# Autodesk Inventor assembly: Sheet_Assembly
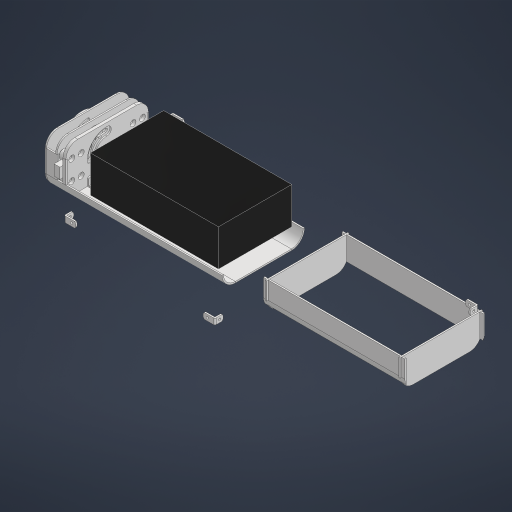
[picture p0: Inventor's stored thumbnail of the model, 512x512]
Saved by Autodesk Inventor 2024 (Build 280153000, 153)
## iProperties
Created: 2024-02-24
Part Number: Sheet_Assembly
Document SubType Name: Assembly
Designer: calvi
Author: calvi
## Documents named in this file (15)
- C:\Users\calvi\OneDrive\Robocup Rescue\Chassis\Battery Drawer\Sheet_Assembly.iam
- C:\Users\calvi\OneDrive\Robocup Rescue\Chassis\Battery Drawer\Sheet.ipt
- C:\Users\calvi\OneDrive\Robocup Rescue\Chassis\Battery Drawer\Plate_middle.ipt
- C:\Users\calvi\OneDrive\Robocup Rescue\Chassis\Battery Drawer\Plate_back.ipt
- C:\Users\calvi\OneDrive\Robocup Rescue\Chassis\Battery Drawer\Crank.ipt
- C:\Users\calvi\OneDrive\Robocup Rescue\Chassis\Battery Drawer\Peg.ipt
- C:\Users\calvi\OneDrive\Robocup Rescue\Chassis\Battery Drawer\Handle.ipt
- C:\Users\calvi\OneDrive\Robocup Rescue\Chassis\Battery Drawer\Slider1.ipt
- Slider1.ipt
- C:\Users\calvi\OneDrive\Robocup Rescue\Chassis\Battery Drawer\Slider2.ipt
- C:\Users\calvi\OneDrive\Robocup Rescue\Chassis\Battery Drawer\6389K345_Light Duty Dry-Running Nylon Sleeve Bearing\6389K345_Light Duty Dry-Running Nylon Sleeve Bearing.ipt
- C:\Users\calvi\OneDrive\Robocup Rescue\Chassis\Battery Drawer\Zinc-Plated Steel Corner Bracket3\Zinc-Plated Steel Corner Bracket3.ipt
- C:\Users\calvi\OneDrive\Robocup Rescue\Chassis\Electronics Box\EBox-Parts\MainBattery.ipt
- MainBattery-E.ipt
- C:\Users\calvi\OneDrive\Robocup Rescue\Chassis\Battery Drawer\BatteryHolder\Battery_Holder_Assembly.iam
## Components (27 placed, 12 different names)
1. Sheet:1 — Mate:1, Mate:2, Mate:3, Mate:4, Mate:5, Mate:10, Mate:12, Mate:13, Mate:15, Rotational:9, Mate:18, Mate:19, Mate:20, Mate:21, Mate:27, Mate:28
2. Plate_middle:1 — Mate:1, Mate:2, Mate:3, Rotational:1, Rotational:2, Rotational:3, Rotational:4, Rotational:5, Rotational:6, Rotational:7, Rotational:8, Mate:6, Flush:1, Mate:7, Flush:2, Mate:16, Mate:17
3. Plate_back:1 — Mate:4, Mate:5, Rigid:1, Mate:11, Mate:14
4. Crank:1 — Rigid:10, Rotational:9, Cylindrical:1, Cylindrical:2
5. Peg:1 — Slider:2, Cylindrical:1
6. Peg:2 — Slider:1, Cylindrical:2
7. Handle:1 — Rigid:10
8. Slider1:1 — Mate:6, Flush:1, Slider:2
9. Slider2:1 — Mate:7, Flush:2, Slider:1
10. MainBattery-E:2 — Mate:25
11. Battery_Holder_Assembly:1 [sub-assembly] — Mate:25, Mate:27, Mate:28, Mate:29, Mate:30
12. Zinc-Plated Steel Corner Bracket3:5
13. Zinc-Plated Steel Corner Bracket3:6
14. Zinc-Plated Steel Corner Bracket3:7
15. Zinc-Plated Steel Corner Bracket3:8 — Mate:29, Mate:30
16. 6389K345_Light Duty Dry-Running Nylon Sleeve Bearing:8 — Rotational:8
17. 6389K345_Light Duty Dry-Running Nylon Sleeve Bearing:7 — Rotational:7
18. 6389K345_Light Duty Dry-Running Nylon Sleeve Bearing:6 — Rotational:5
19. 6389K345_Light Duty Dry-Running Nylon Sleeve Bearing:5 — Rotational:6, Rigid:1
20. 6389K345_Light Duty Dry-Running Nylon Sleeve Bearing:4 — Rotational:4
21. 6389K345_Light Duty Dry-Running Nylon Sleeve Bearing:3 — Rotational:3
22. 6389K345_Light Duty Dry-Running Nylon Sleeve Bearing:2 — Rotational:2
23. 6389K345_Light Duty Dry-Running Nylon Sleeve Bearing:1 — Rotational:1
24. Zinc-Plated Steel Corner Bracket3:4 — Mate:17, Mate:18, Mate:21
25. Zinc-Plated Steel Corner Bracket3:3 — Mate:16, Mate:19, Mate:20
26. Zinc-Plated Steel Corner Bracket3:2 — Mate:13, Mate:14, Mate:15
27. Zinc-Plated Steel Corner Bracket3:1 — Mate:10, Mate:11, Mate:12
## Relationships (41: Mate 24, RevoluteJoint 9, Flush 2, WeldJoint 2, TranslationJoint 2, CylindricalJoint 2)
- Mate:1: Sheet:1 ↔ Plate_middle:1
- Mate:2: Sheet:1 ↔ Plate_middle:1
- Mate:3 (19.177 mm): Sheet:1 ↔ Plate_middle:1
- Mate:4: Sheet:1 ↔ Plate_back:1
- Mate:5: Sheet:1 ↔ Plate_back:1
- Rotational:1 [RevoluteJoint]: Plate_middle:1 ↔ 6389K345_Light Duty Dry-Running Nylon Sleeve Bearing:1
- Rotational:2 [RevoluteJoint]: Plate_middle:1 ↔ 6389K345_Light Duty Dry-Running Nylon Sleeve Bearing:2
- Rotational:3 [RevoluteJoint]: Plate_middle:1 ↔ 6389K345_Light Duty Dry-Running Nylon Sleeve Bearing:3
- Rotational:4 [RevoluteJoint]: Plate_middle:1 ↔ 6389K345_Light Duty Dry-Running Nylon Sleeve Bearing:4
- Rotational:5 [RevoluteJoint]: Plate_middle:1 ↔ 6389K345_Light Duty Dry-Running Nylon Sleeve Bearing:6
- Rotational:6 [RevoluteJoint]: Plate_middle:1 ↔ 6389K345_Light Duty Dry-Running Nylon Sleeve Bearing:5
- Rotational:7 [RevoluteJoint]: Plate_middle:1 ↔ 6389K345_Light Duty Dry-Running Nylon Sleeve Bearing:7
- Rotational:8 [RevoluteJoint]: Plate_middle:1 ↔ 6389K345_Light Duty Dry-Running Nylon Sleeve Bearing:8
- Mate:6: Plate_middle:1 ↔ Slider1:1
- Flush:1 (-11.43 mm): Plate_middle:1 ↔ Slider1:1
- Mate:7: Plate_middle:1 ↔ Slider2:1
- Flush:2 (-11.43 mm): Plate_middle:1 ↔ Slider2:1
- Rigid:1 [WeldJoint]: Plate_back:1 ↔ 6389K345_Light Duty Dry-Running Nylon Sleeve Bearing:5
- Mate:10: Sheet:1 ↔ Zinc-Plated Steel Corner Bracket3:1
- Mate:11: Plate_back:1 ↔ Zinc-Plated Steel Corner Bracket3:1
- Mate:12 (43.18 mm): Sheet:1 ↔ Zinc-Plated Steel Corner Bracket3:1
- Mate:13: Sheet:1 ↔ Zinc-Plated Steel Corner Bracket3:2
- Mate:14: Plate_back:1 ↔ Zinc-Plated Steel Corner Bracket3:2
- Mate:15 (43.18 mm): Sheet:1 ↔ Zinc-Plated Steel Corner Bracket3:2
- Rigid:10 [WeldJoint]: Crank:1 ↔ Handle:1
- Rotational:9 [RevoluteJoint]: Sheet:1 ↔ Crank:1
- Slider:1 [TranslationJoint] (-6.35 mm): Peg:2 ↔ Slider2:1
- Slider:2 [TranslationJoint] (-12.7 mm): Peg:1 ↔ Slider1:1
- Cylindrical:1: Crank:1 ↔ Peg:1
- Cylindrical:2: Crank:1 ↔ Peg:2
- Mate:16: Plate_middle:1 ↔ Zinc-Plated Steel Corner Bracket3:3
- Mate:17: Plate_middle:1 ↔ Zinc-Plated Steel Corner Bracket3:4
- Mate:18: Sheet:1 ↔ Zinc-Plated Steel Corner Bracket3:4
- Mate:19: Sheet:1 ↔ Zinc-Plated Steel Corner Bracket3:3
- Mate:20 (43.18 mm): Sheet:1 ↔ Zinc-Plated Steel Corner Bracket3:3
- Mate:21 (43.18 mm): Sheet:1 ↔ Zinc-Plated Steel Corner Bracket3:4
- Mate:25 (3.81 mm): MainBattery-E:2 ↔ Battery_Holder_Assembly:1
- Mate:27: Sheet:1 ↔ Battery_Holder_Assembly:1
- Mate:28: Sheet:1 ↔ Battery_Holder_Assembly:1
- Mate:29: Battery_Holder_Assembly:1 ↔ Zinc-Plated Steel Corner Bracket3:8
- Mate:30: Battery_Holder_Assembly:1 ↔ Zinc-Plated Steel Corner Bracket3:8
